# Autodesk Inventor assembly: idler
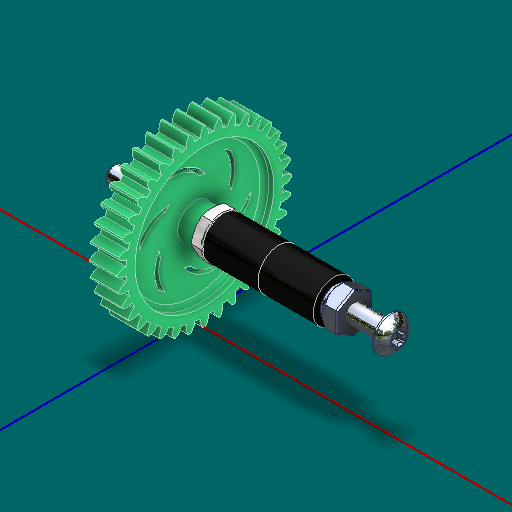
[picture p0: Inventor's stored thumbnail of the model, 512x512]
Saved by Autodesk Inventor 2025 (Build 290162000, 162)
## iProperties
Created: 2024-08-21
Part Number: idler
Document SubType Name: Assembly
Designer: averey
Author: averey
## Documents named in this file (11)
- C:\Users\avere\vex_robotics_high_stakes\hardware\cad\bots\ENIGMA\chassis\drivetrain\drivebay\idler.iam
- C:\Users\avere\vex_robotics_high_stakes\hardware\cad\VEX-CAD-Inventor\Motion\Gears\LS 36T Gear.ipt
- C:\Users\avere\vex_robotics_high_stakes\hardware\cad\VEX-CAD-Inventor\Motion\Spacers\Spacer Nylon .375 OD.ipt
- C:\Users\avere\vex_robotics_high_stakes\hardware\cad\VEX-CAD-Inventor\Motion\Spacers\Spacer Nylon .375 OD\NSpacer .375 OD x .500.ipt
- C:\Users\avere\vex_robotics_high_stakes\hardware\cad\VEX-CAD-Inventor\Motion\Spacers\Washer Steel\SWasher .375 OD x .015625.ipt
- C:\Users\avere\vex_robotics_high_stakes\hardware\cad\VEX-CAD-Inventor\Motion\Spacers\Washer Steel.ipt
- C:\Users\avere\vex_robotics_high_stakes\hardware\cad\VEX-CAD-Inventor\Structure\Hardware\Nut Thin Nylock.ipt
- C:\Users\avere\vex_robotics_high_stakes\hardware\cad\VEX-CAD-Inventor\Structure\Hardware\Screw Steel - Star\SScrew Star Smooth 2.500.ipt
- C:\Users\avere\vex_robotics_high_stakes\hardware\cad\VEX-CAD-Inventor\Structure\Hardware\Screw Steel - Star.ipt
- C:\Users\avere\vex_robotics_high_stakes\hardware\cad\VEX-CAD-Inventor\Structure\Hardware\Nut Nylon\Nut Nylon - White.ipt
- C:\Users\avere\vex_robotics_high_stakes\hardware\cad\VEX-CAD-Inventor\Structure\Hardware\Nut Nylon.ipt
## Components (7 placed, 6 different names)
1. LS 36T Gear:1 — Insert:5, Insert:6
2. NSpacer .375 OD x .500:2 — Insert:1, Insert:2
3. NSpacer .375 OD x .500:3 — Insert:1, Insert:3
4. SWasher .375 OD x .015625:1 — Insert:2, Insert:5
5. Nut Thin Nylock:1 — Insert:3, Insert:4
6. SScrew Star Smooth 2.500:1 — Insert:4
7. Nut Nylon - White:1 — Insert:6
## Relationships (6: Insert 6)
- Insert:1: NSpacer .375 OD x .500:2 ↔ NSpacer .375 OD x .500:3
- Insert:2: NSpacer .375 OD x .500:2 ↔ SWasher .375 OD x .015625:1
- Insert:3: NSpacer .375 OD x .500:3 ↔ Nut Thin Nylock:1
- Insert:4 (7.9375 mm): Nut Thin Nylock:1 ↔ SScrew Star Smooth 2.500:1
- Insert:5 (2.3813 mm): LS 36T Gear:1 ↔ SWasher .375 OD x .015625:1
- Insert:6: LS 36T Gear:1 ↔ Nut Nylon - White:1
